# Autodesk Inventor assembly: towerbottom2.3
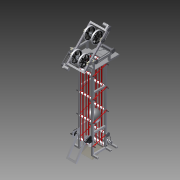
[picture p0: Inventor's stored thumbnail of the model, 180x180]
Saved by Autodesk Inventor 2011 SP1 (Build 150282100, 282)
## iProperties
Created: 2012-01-19
Part Number: towerbottom2.3
Document SubType Name: Assembly
Designer: Christopher
Author: Christopher
## Documents named in this file (27)
- C:\Users\Christopher\Documents\Christopher\FIRST\Inventor files\2012\tower bottom second design\towerbottom2.3.iam
- C:\Users\Christopher\Documents\Christopher\FIRST\Inventor files\2012\tower first design\towertallbackthing.ipt
- C:\Users\Christopher\Documents\Christopher\FIRST\Inventor files\2012\tower bottom second design\tower horizontal brace 17.5in.ipt
- C:\Users\Christopher\Documents\Christopher\FIRST\Inventor files\2012\tower bottom second design\towermiddle8inbrace.ipt
- C:\Users\Christopher\Documents\Christopher\FIRST\Inventor files\2012\tower bottom second design\towerside4.5inbrace.ipt
- C:\Users\Christopher\Documents\Christopher\FIRST\Inventor files\2011\Kit of Parts\motors\Motors_Denso_262100-3030.ipt
- C:\Users\Christopher\Documents\Christopher\FIRST\Inventor files\2011\Kit of Parts\motors\Motors_Denso_262100-3040.ipt
- C:\Users\Christopher\Documents\Christopher\FIRST\Inventor files\2012\tower bottom second design\window motor plate.ipt
- C:\Users\Christopher\Documents\Christopher\FIRST\Inventor files\2012\tower bottom second design\ramp1.ipt
- C:\Users\Christopher\Documents\Christopher\FIRST\Inventor files\2011\Kit of Parts\motors\Motors_Pelham Plastics_Denso-6.ipt
- C:\Users\Christopher\Documents\Christopher\FIRST\Inventor files\2012\tower bottom second design\bambar 12 in.ipt
- C:\Users\Christopher\Documents\Christopher\FIRST\Inventor files\2012\tower bottom second design\bambar 8.5 inch.ipt
- C:\Users\Christopher\Documents\Christopher\FIRST\Inventor files\2012\tower bottom second design\11in axle.ipt
- C:\Users\Christopher\Documents\Christopher\FIRST\Inventor files\2012\tower bottom second design\axlebracetopvc.ipt
- C:\Users\Christopher\Documents\Christopher\FIRST\Inventor files\2012\tower bottom second design\8 in pvc roller 1.379.ipt
- C:\Users\Christopher\Documents\Christopher\FIRST\Inventor files\2012\tower bottom second design\13 in axle.ipt
- C:\Users\Christopher\Documents\Christopher\FIRST\Inventor files\2012\tower bottom second design\2.5ingear proxy.ipt
- C:\Users\Christopher\Documents\Christopher\FIRST\Inventor files\2012\tower bottom second design\tower horizontal brace 17.5in_CPY.ipt
- C:\Users\Christopher\Documents\Christopher\FIRST\Inventor files\2012\tower bottom second design\proxycimulator775.ipt
- C:\Users\Christopher\Documents\Christopher\FIRST\Inventor files\2012\tower bottom second design\proxy chain 1.ipt
- C:\Users\Christopher\Documents\Christopher\FIRST\Inventor files\2012\tower bottom second design\towertallfrontthing.ipt
- C:\Users\Christopher\Documents\Christopher\FIRST\Inventor files\2012\tower bottom second design\polycord cross proxy.ipt
- C:\Users\Christopher\Documents\Christopher\FIRST\Inventor files\2012\4 wheel kicker version 1\proxy 775 motor.ipt
- C:\Users\Christopher\Documents\Christopher\FIRST\Inventor files\2012\4 wheel kicker version 1\game ball.ipt
- C:\Users\Christopher\Documents\Christopher\FIRST\Inventor files\2012\tower bottom second design\7in polycord loop.ipt
- C:\Users\Christopher\Documents\Christopher\FIRST\Inventor files\2012\tower bottom second design\roller.iam
- C:\Users\Christopher\Documents\Christopher\FIRST\Inventor files\2012\shooter design 2\vertical shooter 1.3.iam
## Components (60 placed, 26 different names)
1. towertallbackthing:3 — Mate:5, Flush:8, Flush:9, Insert:9, Insert:12, Insert:15, Insert:16, Insert:29, Insert:30, Insert:31, Insert:35, Insert:36, Insert:37, Mate:36, Flush:41
2. towertallbackthing:4 — Mate:6, Flush:10, Flush:11, Insert:7, Insert:8, Insert:13, Insert:38, Insert:39, Insert:40
3. tower horizontal brace 17.5in:2 — Mate:2, Flush:3, Flush:4, Mate:5, Flush:8, Flush:9, Mate:6, Flush:10, Flush:11, Flush:12, Mate:7, Flush:13, Mate:12, Flush:19, Flush:28, Flush:29, Mate:23
4. towermiddle8inbrace:1 — Mate:2, Flush:3, Flush:4, Mate:11, Flush:15, Flush:16, Mate:13, Flush:32, Mate:35, Mate:37
5. towermiddle8inbrace:2 — Flush:12, Mate:7, Flush:13, Mate:8, Flush:14, Mate:18, Flush:36, Mate:30, Mate:33, Mate:34
6. towerside4.5inbrace:1 — Mate:11, Flush:15, Flush:16, Mate:15, Mate:25, Flush:33, Mate:27
7. towerside4.5inbrace:2 — Mate:8, Flush:14, Mate:17, Mate:28, Flush:35
8. Motors_Denso_262100-3030:1 — Insert:1, Insert:4
9. Motors_Denso_262100-3040:1 — Insert:2, Insert:3
10. window motor plate:1 — Insert:1, Mate:15, Mate:26, Flush:34, Mate:27
11. window motor plate:2 — Mate:17, Insert:2, Mate:18, Mate:29, Mate:30, Flush:37
12. ramp1:1 — Mate:12, Flush:19, Mate:13
13. Motors_Pelham Plastics_Denso-6:1 — Insert:3, Insert:5, Insert:6
14. Motors_Pelham Plastics_Denso-6:2 — Insert:4
15. bambar 12 in:1 — Flush:23, Mate:19, Flush:24
16. bambar 12 in:2 — Mate:20, Flush:25, Flush:26, Insert:5, Insert:6
17. bambar 8.5 inch:1 — Flush:23, Mate:19, Flush:24, Mate:20, Flush:25, Flush:26
18. 11in axle:1 — Insert:7
19. axlebracetopvc:1 — Insert:9
20. axlebracetopvc:2 — Insert:8, Insert:10
21. 8 in pvc roller 1.379:1 — Insert:10
22. axlebracetopvc:3 — Insert:13
23. axlebracetopvc:4 — Insert:12, Insert:14
24. 8 in pvc roller 1.379:2 — Insert:14, Insert:25, Insert:26, Insert:27, Insert:28
25. 13 in axle:1 — Insert:15
26. 2.5ingear proxy:1 — Insert:16, Insert:17
27. tower horizontal brace 17.5in_CPY:1 — Flush:28, Flush:29, Mate:23, Mate:24, Flush:30, Flush:31
28. proxycimulator775:1 — Mate:24, Flush:30, Flush:31, Insert:23
29. proxy chain 1:1 — Insert:17
30. towertallfrontthing:1 — Mate:25, Flush:32, Flush:33, Mate:26, Flush:34, Insert:18, Insert:20, Insert:24, Insert:32, Insert:33, Insert:34, Flush:42, Mate:38, Mate:39, Mate:40, Mate:41
31. towertallfrontthing:2 — Mate:28, Flush:35, Flush:36, Mate:29, Flush:37, Insert:19, Insert:22, Mate:31, Flush:38, Mate:32, Flush:39, Flush:40
32. 8 in pvc roller 1.379:3 — Insert:21
33. 13 in axle:2 — Insert:18
34. axlebracetopvc:5 — Insert:20, Insert:21
35. axlebracetopvc:6 — Insert:19
36. polycord cross proxy:1 — Insert:22
37. proxy 775 motor:1 — Insert:23
38. game ball:1
39. polycord cross proxy:2 — Insert:24
40. 7in polycord loop:1 — Insert:25
41. 7in polycord loop:2 — Insert:26
42. 7in polycord loop:3 — Insert:27
43. 7in polycord loop:4 — Insert:28
44. roller:1 [sub-assembly] — Insert:30
45. roller:2 [sub-assembly] — Insert:29
46. roller:3 [sub-assembly] — Insert:31
47. roller:4 [sub-assembly] — Insert:34
48. roller:5 [sub-assembly] — Insert:32
49. roller:6 [sub-assembly] — Insert:33
50. polycord cross proxy:3 — Insert:35
51. polycord cross proxy:4 — Insert:36
52. polycord cross proxy:5 — Insert:37
53. polycord cross proxy:6 — Insert:38
54. polycord cross proxy:7 — Insert:39
55. polycord cross proxy:8 — Insert:40
56. towermiddle8inbrace:3 — Mate:32, Flush:39, Mate:33
57. towermiddle8inbrace:4 — Mate:31, Flush:38, Mate:34, Flush:40
58. towermiddle8inbrace:5 — Mate:37, Flush:42, Mate:38
59. towermiddle8inbrace:6 — Mate:35, Mate:36, Flush:41
60. vertical shooter 1.3:1 [sub-assembly] — Mate:39, Mate:40, Mate:41
## Relationships (102: Insert 39, Mate 32, Flush 31)
- Mate:2: tower horizontal brace 17.5in:2 ↔ towermiddle8inbrace:1
- Flush:3: tower horizontal brace 17.5in:2 ↔ towermiddle8inbrace:1
- Flush:4 (-88.9 mm): tower horizontal brace 17.5in:2 ↔ towermiddle8inbrace:1
- Mate:5: towertallbackthing:3 ↔ tower horizontal brace 17.5in:2
- Flush:8: towertallbackthing:3 ↔ tower horizontal brace 17.5in:2
- Flush:9 (88.9 mm): towertallbackthing:3 ↔ tower horizontal brace 17.5in:2
- Mate:6: towertallbackthing:4 ↔ tower horizontal brace 17.5in:2
- Flush:10: towertallbackthing:4 ↔ tower horizontal brace 17.5in:2
- Flush:11 (88.9 mm): towertallbackthing:4 ↔ tower horizontal brace 17.5in:2
- Flush:12: tower horizontal brace 17.5in:2 ↔ towermiddle8inbrace:2
- Mate:7: tower horizontal brace 17.5in:2 ↔ towermiddle8inbrace:2
- Flush:13 (-88.9 mm): tower horizontal brace 17.5in:2 ↔ towermiddle8inbrace:2
- Mate:8: towermiddle8inbrace:2 ↔ towerside4.5inbrace:2
- Flush:14: towermiddle8inbrace:2 ↔ towerside4.5inbrace:2
- Mate:11: towermiddle8inbrace:1 ↔ towerside4.5inbrace:1
- Flush:15: towermiddle8inbrace:1 ↔ towerside4.5inbrace:1
- Flush:16: towermiddle8inbrace:1 ↔ towerside4.5inbrace:1
- Insert:1: Motors_Denso_262100-3030:1 ↔ window motor plate:1
- Mate:12: tower horizontal brace 17.5in:2 ↔ ramp1:1
- Flush:19: tower horizontal brace 17.5in:2 ↔ ramp1:1
- Mate:13: towermiddle8inbrace:1 ↔ ramp1:1
- Mate:15 (203.2 mm): towerside4.5inbrace:1 ↔ window motor plate:1
- Mate:17 (203.2 mm): towerside4.5inbrace:2 ↔ window motor plate:2
- Insert:2: Motors_Denso_262100-3040:1 ↔ window motor plate:2
- Mate:18 (203.2 mm): towermiddle8inbrace:2 ↔ window motor plate:2
- Insert:3: Motors_Denso_262100-3040:1 ↔ Motors_Pelham Plastics_Denso-6:1
- Insert:4: Motors_Denso_262100-3030:1 ↔ Motors_Pelham Plastics_Denso-6:2
- Flush:23: bambar 12 in:1 ↔ bambar 8.5 inch:1
- Mate:19: bambar 12 in:1 ↔ bambar 8.5 inch:1
- Flush:24: bambar 12 in:1 ↔ bambar 8.5 inch:1
- Mate:20: bambar 12 in:2 ↔ bambar 8.5 inch:1
- Flush:25: bambar 12 in:2 ↔ bambar 8.5 inch:1
- Flush:26: bambar 12 in:2 ↔ bambar 8.5 inch:1
- Insert:5: Motors_Pelham Plastics_Denso-6:1 ↔ bambar 12 in:2
- Insert:6: Motors_Pelham Plastics_Denso-6:1 ↔ bambar 12 in:2
- Insert:7 (-12.7 mm): towertallbackthing:4 ↔ 11in axle:1
- Insert:8: towertallbackthing:4 ↔ axlebracetopvc:2
- Insert:9: towertallbackthing:3 ↔ axlebracetopvc:1
- Insert:10: axlebracetopvc:2 ↔ 8 in pvc roller 1.379:1
- Insert:12: towertallbackthing:3 ↔ axlebracetopvc:4
- Insert:13: towertallbackthing:4 ↔ axlebracetopvc:3
- Insert:14: axlebracetopvc:4 ↔ 8 in pvc roller 1.379:2
- Insert:15 (-38.1 mm): towertallbackthing:3 ↔ 13 in axle:1
- Insert:16 (6.35 mm): towertallbackthing:3 ↔ 2.5ingear proxy:1
- Flush:28: tower horizontal brace 17.5in:2 ↔ tower horizontal brace 17.5in_CPY:1
- Flush:29: tower horizontal brace 17.5in:2 ↔ tower horizontal brace 17.5in_CPY:1
- Mate:23 (76.2 mm): tower horizontal brace 17.5in:2 ↔ tower horizontal brace 17.5in_CPY:1
- Mate:24: tower horizontal brace 17.5in_CPY:1 ↔ proxycimulator775:1
- Flush:30 (88.9 mm): tower horizontal brace 17.5in_CPY:1 ↔ proxycimulator775:1
- Flush:31: tower horizontal brace 17.5in_CPY:1 ↔ proxycimulator775:1
- Insert:17: 2.5ingear proxy:1 ↔ proxy chain 1:1
- Mate:25: towerside4.5inbrace:1 ↔ towertallfrontthing:1
- Flush:32: towermiddle8inbrace:1 ↔ towertallfrontthing:1
- Flush:33: towerside4.5inbrace:1 ↔ towertallfrontthing:1
- Mate:26: window motor plate:1 ↔ towertallfrontthing:1
- Flush:34: window motor plate:1 ↔ towertallfrontthing:1
- Mate:27 (203.2 mm): towerside4.5inbrace:1 ↔ window motor plate:1
- Mate:28: towerside4.5inbrace:2 ↔ towertallfrontthing:2
- Flush:35: towerside4.5inbrace:2 ↔ towertallfrontthing:2
- Flush:36: towermiddle8inbrace:2 ↔ towertallfrontthing:2
- Mate:29: window motor plate:2 ↔ towertallfrontthing:2
- Mate:30 (203.2 mm): towermiddle8inbrace:2 ↔ window motor plate:2
- Flush:37: window motor plate:2 ↔ towertallfrontthing:2
- Insert:18 (-38.1 mm): towertallfrontthing:1 ↔ 13 in axle:2
- Insert:19: towertallfrontthing:2 ↔ axlebracetopvc:6
- Insert:20: towertallfrontthing:1 ↔ axlebracetopvc:5
- Insert:21: 8 in pvc roller 1.379:3 ↔ axlebracetopvc:5
- Insert:22: towertallfrontthing:2 ↔ polycord cross proxy:1
- Insert:23: proxycimulator775:1 ↔ proxy 775 motor:1
- Insert:24: towertallfrontthing:1 ↔ polycord cross proxy:2
- Insert:25 (25.4 mm): 8 in pvc roller 1.379:2 ↔ 7in polycord loop:1
- Insert:26 (76.2 mm): 8 in pvc roller 1.379:2 ↔ 7in polycord loop:2
- Insert:27 (127 mm): 8 in pvc roller 1.379:2 ↔ 7in polycord loop:3
- Insert:28 (177.8 mm): 8 in pvc roller 1.379:2 ↔ 7in polycord loop:4
- Insert:29 (-38.1 mm): towertallbackthing:3 ↔ roller:2
- Insert:30 (-38.1 mm): towertallbackthing:3 ↔ roller:1
- Insert:31 (-38.1 mm): towertallbackthing:3 ↔ roller:3
- Insert:32 (-38.1 mm): towertallfrontthing:1 ↔ roller:5
- Insert:33 (-38.1 mm): towertallfrontthing:1 ↔ roller:6
- Insert:34 (-38.1 mm): towertallfrontthing:1 ↔ roller:4
- Insert:35: towertallbackthing:3 ↔ polycord cross proxy:3
- Insert:36: towertallbackthing:3 ↔ polycord cross proxy:4
- Insert:37: towertallbackthing:3 ↔ polycord cross proxy:5
- Insert:38: towertallbackthing:4 ↔ polycord cross proxy:6
- Insert:39: towertallbackthing:4 ↔ polycord cross proxy:7
- Insert:40: towertallbackthing:4 ↔ polycord cross proxy:8
- Mate:31: towertallfrontthing:2 ↔ towermiddle8inbrace:4
- Flush:38: towertallfrontthing:2 ↔ towermiddle8inbrace:4
- Mate:32: towertallfrontthing:2 ↔ towermiddle8inbrace:3
- Flush:39: towertallfrontthing:2 ↔ towermiddle8inbrace:3
- Mate:33 (914.4 mm): towermiddle8inbrace:2 ↔ towermiddle8inbrace:3
- Mate:34 (304.8 mm): towermiddle8inbrace:2 ↔ towermiddle8inbrace:4
- Flush:40: towertallfrontthing:2 ↔ towermiddle8inbrace:4
- Mate:35 (304.8 mm): towermiddle8inbrace:1 ↔ towermiddle8inbrace:6
- Mate:36: towertallbackthing:3 ↔ towermiddle8inbrace:6
- Flush:41: towertallbackthing:3 ↔ towermiddle8inbrace:6
- Mate:37 (914.4 mm): towermiddle8inbrace:1 ↔ towermiddle8inbrace:5
- Flush:42: towertallfrontthing:1 ↔ towermiddle8inbrace:5
- Mate:38: towertallfrontthing:1 ↔ towermiddle8inbrace:5
- Mate:39: towertallfrontthing:1 ↔ vertical shooter 1.3:1
- Mate:40 (12.7 mm): towertallfrontthing:1 ↔ vertical shooter 1.3:1
- Mate:41: towertallfrontthing:1 ↔ vertical shooter 1.3:1
